# Autodesk Inventor assembly: 링크
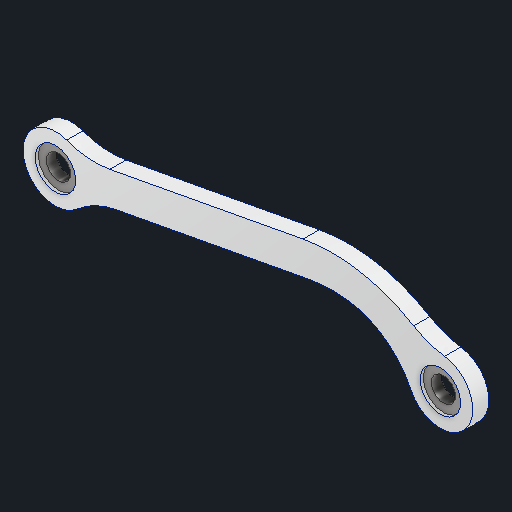
[picture p0: Inventor's stored thumbnail of the model, 512x512]
Saved by Autodesk Inventor 2027.1 (Build 311270010, 270A)
## iProperties
Created: 2026-08-20
Part Number: 링크
Document SubType Name: Assembly
Designer: moieboy9999
Mass: 12.2306 g
Surface Area: 36.0563 cm^2
Volume: 4.04043 cm^3
Density: 3.02705 g/cm^3
Author: moieboy9999
## Documents named in this file (3)
- D:\micro_dog_cad\다리\프레임\링크.iam
- D:\micro_dog_cad\다리\프레임\링크.ipt
- D:\micro_dog_cad\부품\작은베어링.ipt
## Components (3 placed, 2 different names)
1. 링크:1 — 메이트:1, 플러쉬:1, 메이트:2, 플러쉬:2
2. 작은베어링:1 — 메이트:2, 플러쉬:2
3. 작은베어링:2 — 메이트:1, 플러쉬:1
## Relationships (4: Mate 2, Flush 2)
- 메이트:1 [Mate]: 링크:1 ↔ 작은베어링:2
- 플러쉬:1 [Flush] (0.75 mm): 링크:1 ↔ 작은베어링:2
- 메이트:2 [Mate]: 링크:1 ↔ 작은베어링:1
- 플러쉬:2 [Flush] (0.75 mm): 링크:1 ↔ 작은베어링:1
